# Autodesk Inventor assembly: Rebreather_TMH_Clinical_Test
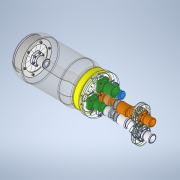
[picture p0: Inventor's stored thumbnail of the model, 180x180]
Saved by Autodesk Inventor 2020 (Build 240168000, 168)
## iProperties
Created: 2021-06-26
Part Number: Rebreather_TMH_Clinical_Test
Document SubType Name: Assembly
Designer: Workshop
Author: Workshop
## Documents named in this file (36)
- D:\Daya 2\Oxy\Bottle D 4 TMH Clinical\3d Files\Rebreather_TMH_Clinical_Test.iam
- D:\Daya 2\Oxy\Bottle D 4 TMH Clinical\3d Files\Container(Sunpet_2L).ipt
- D:\Daya 2\Oxy\Bottle D 4 TMH Clinical\3d Files\Container_Lid(Sunpet_2L).ipt
- D:\Daya 2\Oxy\Bottle D 4 TMH Clinical\3d Files\Bottom_Plate_For_Valve.ipt
- D:\Daya 2\Oxy\Bottle D 4 TMH Clinical\3d Files\Middle_Plate_For_Valve.ipt
- D:\Daya 2\Oxy\Bottle D 4 TMH Clinical\3d Files\Top_Plate_For_Valve.ipt
- C:\Users\Workshop\Documents\Inventor\Content Center Files\R2020\en-US\BS 4168(8)\BS 4168 - M3 x 16(7).ipt
- D:\Daya 2\Oxy\Bottle D 4 TMH Clinical\3d Files\M3_Nylon_Nut.ipt
- D:\Daya 2\Oxy\Bottle D 4 TMH Clinical\3d Files\Silicon_Valve.ipt
- D:\Daya 2\Oxy\Bottle D 4 TMH Clinical\3d Files\Net_Filter.ipt
- D:\Daya 2\Oxy\Bottle D 4 TMH Clinical\3d Files\Net_Retainer.ipt
- D:\Daya 2\Oxy\Bottle D 4 TMH Clinical\3d Files\22M_Airbag_Port_Green.ipt
- D:\Daya 2\Oxy\Bottle D 4 TMH Clinical\3d Files\22M_Exhalation_Port_Orange.ipt
- D:\Daya 2\Oxy\Bottle D 4 TMH Clinical\3d Files\22M_Inhalation_Port_Blue.ipt
- D:\Daya 2\Oxy\Bottle D 4 TMH Clinical\3d Files\22M_PEEP_Port_Female_Green.ipt
- D:\Daya 2\Oxy\Bottle D 4 TMH Clinical\3d Files\22M_Venturi_Port_White.ipt
- D:\Daya 2\Oxy\Bottle D 4 TMH Clinical\3d Files\22M_Diffuser_Port_Sq_Black.ipt
- D:\Daya 2\Oxy\Bottle D 4 TMH Clinical\3d Files\Diffuser_Bottom_Cover.ipt
- D:\Daya 2\Oxy\Bottle D 4 TMH Clinical\3d Files\Diffuser_Filter_Holder.ipt
- D:\Daya 2\Oxy\Bottle D 4 TMH Clinical\3d Files\Diffuser_Top_Cover.ipt
- D:\Daya 2\Oxy\Bottle D 4 TMH Clinical\3d Files\Filter.ipt
- D:\Daya 2\Oxy\Bottle D 4 TMH Clinical\3d Files\22M_Diffuser_Port_Hex_White.ipt
- C:\Users\Workshop\Documents\Inventor\Content Center Files\R2020\en-US\ANSI B18.3.1M(6)\ANSI B18.3.1M - M3x0.5 x 16(1).ipt
- C:\Users\Workshop\Documents\Inventor\Content Center Files\R2020\en-US\ANSI B18.3.1M(6)\ANSI B18.3.1M - M3x0.5 x 45(1).ipt
- D:\Daya 2\Oxy\Bottle D 4 TMH Clinical\3d Files\Connecting_Pipe.ipt
- D:\Daya 2\Oxy\Bottle D 4 TMH Clinical\3d Files\Standalone_Valve_Spacer_Plate.ipt
- D:\Daya 2\Oxy\Bottle D 4 TMH Clinical\3d Files\Standalone_Valve_Cover_Plate.ipt
- D:\Daya 2\Oxy\Bottle D 4 TMH Clinical\3d Files\Standalone_Valve_Base_Plate.ipt
- C:\Users\Workshop\Documents\Inventor\Content Center Files\R2020\en-US\ISO 7091\ISO 7091 - ST 3 - 100 HV.ipt
- C:\Users\Workshop\Documents\Inventor\Content Center Files\R2020\en-US\ANSI B18.3.1M(6)\ANSI B18.3.1M - M3x0.5 x 12(1).ipt
- D:\Daya 2\Oxy\Bottle D 4 TMH Clinical\3d Files\22M_Standalone_Offset_Port_Hex_Female_White.ipt
- D:\Daya 2\Oxy\Bottle D 4 TMH Clinical\3d Files\22M_Standalone_Offset_Port_Hex_Female_Orange.ipt
- D:\Daya 2\Oxy\Bottle D 4 TMH Clinical\3d Files\22M_Standalone_Port_Hex_Lite_Orange.ipt
- D:\Daya 2\Oxy\Bottle D 4 TMH Clinical\3d Files\22M_Standalone_Port_Hex_Lite_White.ipt
- C:\Users\Workshop\Documents\Inventor\Content Center Files\R2020\en-US\ANSI B18.3.1M(6)\ANSI B18.3.1M - M3x0.5 x 25(1).ipt
- D:\Daya 2\Oxy\Bottle D 4 TMH Clinical\3d Files\22M_Male_Female_Adapter.ipt
## Components (118 placed, 35 different names)
1. Container(Sunpet_2L):1 — Mate:1, Mate:2, Flush:1, Insert:1, Insert:48
2. Container_Lid(Sunpet_2L):1 — Insert:1, Mate:3, Insert:2, Insert:3, Insert:11, Insert:12
3. Bottom_Plate_For_Valve:1 — Insert:2, Insert:3, Insert:4, Insert:5, Insert:10
4. Middle_Plate_For_Valve:1 — Insert:4, Insert:5, Insert:6, Insert:7
5. Top_Plate_For_Valve:1 — Insert:6, Insert:7, Insert:8, Insert:9, Angle:1, Insert:15, Insert:16, Insert:17, Insert:18, Insert:19, Insert:20, Insert:21, Insert:22, Insert:23, Insert:24
6. BS 4168 : Part 8 Hexagon socket countersunk and button head screws - Metric series - Metric M3 x 16:1 — Insert:8
7. M3_Nylon_Nut:1 — Insert:9, Angle:1
8. Silicon_Valve:1 — Insert:10
9. Net_Filter:1 — Insert:11, Insert:12, Insert:13, Insert:14, Insert:54, Insert:55
10. Net_Retainer:1 — Insert:13, Insert:14, Insert:25, Insert:26, Insert:56, Insert:57
11. 22M_Airbag_Port_Green:1 — Insert:23, Insert:24
12. 22M_Exhalation_Port_Orange:1 — Insert:17, Insert:18, Insert:49, Insert:50, Insert:51, Insert:52, Insert:107, Angle:9
13. 22M_Inhalation_Port_Blue:1 — Insert:21, Insert:22, Angle:5, Insert:58, Insert:59, Insert:60, Insert:61
14. 22M_PEEP_Port_Female_Green:1 — Insert:19, Insert:20
15. 22M_Venturi_Port_White:1 — Insert:15, Insert:16, Insert:106, Angle:8
16. 22M_Diffuser_Port_Sq_Black:1 — Insert:25, Insert:26, Insert:53, Angle:4, Angle:6, Angle:7
17. Diffuser_Bottom_Cover:1 — Insert:31, Mate:4
18. Diffuser_Filter_Holder:1 — Insert:29, Insert:30, Insert:31, Insert:46, Insert:47
19. Diffuser_Top_Cover:1 — Insert:27, Insert:28, Mate:4, Insert:40, Insert:41, Insert:42, Insert:43, Insert:44, Insert:45, Insert:48
20. Filter:1 — Insert:27, Insert:28, Insert:29, Insert:30, Insert:32, Insert:33
21. 22M_Diffuser_Port_Hex_White:1 — Insert:32, Insert:33, Insert:34, Insert:35, Insert:36, Insert:37, Insert:38, Insert:39, Angle:2, Angle:3, Insert:62
22. Forged Socket Head Cap Screw - Metric M3x0.5 x 16:1 — Insert:34
23. Forged Socket Head Cap Screw - Metric M3x0.5 x 16:2 — Insert:35
24. Forged Socket Head Cap Screw - Metric M3x0.5 x 16:3 — Insert:36
25. Forged Socket Head Cap Screw - Metric M3x0.5 x 16:4 — Insert:37
26. Forged Socket Head Cap Screw - Metric M3x0.5 x 16:5 — Insert:38
27. Forged Socket Head Cap Screw - Metric M3x0.5 x 16:6 — Insert:39
28. Forged Socket Head Cap Screw - Metric M3x0.5 x 16:7 — Insert:40
29. Forged Socket Head Cap Screw - Metric M3x0.5 x 16:8 — Insert:41
30. Forged Socket Head Cap Screw - Metric M3x0.5 x 16:9 — Insert:42
31. Forged Socket Head Cap Screw - Metric M3x0.5 x 16:10 — Insert:43
32. Forged Socket Head Cap Screw - Metric M3x0.5 x 16:11 — Insert:44
33. Forged Socket Head Cap Screw - Metric M3x0.5 x 16:12 — Insert:45
34. Forged Socket Head Cap Screw - Metric M3x0.5 x 45:1 — Insert:49
35. Forged Socket Head Cap Screw - Metric M3x0.5 x 45:2 — Insert:50
36. Forged Socket Head Cap Screw - Metric M3x0.5 x 45:3 — Insert:51
37. Forged Socket Head Cap Screw - Metric M3x0.5 x 45:4 — Insert:52
38. Connecting_Pipe:1 — Insert:62
39. Standalone_Valve_Spacer_Plate:1 — Insert:65, Mate:5, Insert:66, Insert:67
40. Standalone_Valve_Cover_Plate:1 — Insert:68, Insert:69, Insert:74, Insert:93, Mate:9
41. Standalone_Valve_Base_Plate:1 — Insert:63, Insert:65, Mate:5, Insert:91, Insert:92
42. Standalone_Valve_Spacer_Plate:2 — Mate:6, Mate:7, Insert:70, Insert:71, Mate:8
43. Standalone_Valve_Cover_Plate:2 — Insert:72, Insert:73, Insert:75, Insert:88, Insert:89
44. Standalone_Valve_Base_Plate:2 — Insert:64, Mate:6, Mate:7, Insert:90
45. Standalone_Valve_Spacer_Plate:3 — Insert:66, Insert:67, Insert:68, Insert:69
46. Standalone_Valve_Spacer_Plate:4 — Insert:70, Insert:71, Insert:72, Insert:73
47. Silicon_Valve:2 — Insert:63
48. Silicon_Valve:3 — Insert:64
49. ISO 7091 ST 3 - 100 HV:1 — Insert:74, Insert:76
50. ISO 7091 ST 3 - 100 HV:2 — Insert:75, Insert:77
51. Forged Socket Head Cap Screw - Metric M3x0.5 x 12:1 — Insert:76
52. Forged Socket Head Cap Screw - Metric M3x0.5 x 12:2 — Insert:77
53. 22M_Standalone_Offset_Port_Hex_Female_White:1 — Insert:93, Mate:9, Mate:10, Angle:8, Mate:11
54. 22M_Standalone_Offset_Port_Hex_Female_Orange:1 — Insert:88, Insert:89, Mate:12, Angle:9, Mate:13
55. 22M_Standalone_Port_Hex_Lite_Orange:1 — Insert:90, Mate:8, Insert:100, Insert:101, Insert:102, Insert:103, Insert:104, Insert:105
56. 22M_Standalone_Port_Hex_Lite_White:1 — Insert:91, Insert:92, Insert:94, Insert:95, Insert:96, Insert:97, Insert:98, Insert:99
57. Forged Socket Head Cap Screw - Metric M3x0.5 x 25:17 — Insert:94
58. Forged Socket Head Cap Screw - Metric M3x0.5 x 25:18 — Insert:95
59. Forged Socket Head Cap Screw - Metric M3x0.5 x 25:19 — Insert:96
60. Forged Socket Head Cap Screw - Metric M3x0.5 x 25:20 — Insert:97
61. Forged Socket Head Cap Screw - Metric M3x0.5 x 25:21 — Insert:98
62. Forged Socket Head Cap Screw - Metric M3x0.5 x 25:22 — Insert:99
63. Forged Socket Head Cap Screw - Metric M3x0.5 x 25:23 — Insert:100
64. Forged Socket Head Cap Screw - Metric M3x0.5 x 25:24 — Insert:101
65. Forged Socket Head Cap Screw - Metric M3x0.5 x 25:25 — Insert:102
66. Forged Socket Head Cap Screw - Metric M3x0.5 x 25:26 — Insert:103
67. Forged Socket Head Cap Screw - Metric M3x0.5 x 25:27 — Insert:104
68. Forged Socket Head Cap Screw - Metric M3x0.5 x 25:28 — Insert:105
69. 22M_Male_Female_Adapter:1 — Insert:106, Mate:10, Mate:11
70. 22M_Male_Female_Adapter:2 — Insert:107, Mate:12, Mate:13
71. M3_Nylon_Nut:2 — Insert:46, Angle:2
72. M3_Nylon_Nut:3 — Insert:47, Angle:3
73. M3_Nylon_Nut:4
74. M3_Nylon_Nut:5
75. M3_Nylon_Nut:6
76. M3_Nylon_Nut:7
77. M3_Nylon_Nut:8
78. M3_Nylon_Nut:9
79. M3_Nylon_Nut:10
80. M3_Nylon_Nut:11
81. M3_Nylon_Nut:12
82. M3_Nylon_Nut:13
83. M3_Nylon_Nut:14 — Insert:53, Angle:4
84. M3_Nylon_Nut:15
85. M3_Nylon_Nut:16
86. M3_Nylon_Nut:17
87. Forged Socket Head Cap Screw - Metric M3x0.5 x 25:1 — Insert:58
88. M3_Nylon_Nut:18 — Insert:54, Angle:5
89. Forged Socket Head Cap Screw - Metric M3x0.5 x 25:2 — Insert:59
90. M3_Nylon_Nut:19 — Insert:55
91. Forged Socket Head Cap Screw - Metric M3x0.5 x 25:4 — Insert:61
92. M3_Nylon_Nut:20 — Insert:57, Angle:7
93. M3_Nylon_Nut:21 — Insert:56, Angle:6
94. Forged Socket Head Cap Screw - Metric M3x0.5 x 25:3 — Insert:60
95. Forged Socket Head Cap Screw - Metric M3x0.5 x 25:5
96. M3_Nylon_Nut:22
97. Forged Socket Head Cap Screw - Metric M3x0.5 x 25:6
98. M3_Nylon_Nut:23
99. Forged Socket Head Cap Screw - Metric M3x0.5 x 25:7
100. M3_Nylon_Nut:24
101. M3_Nylon_Nut:25
102. Forged Socket Head Cap Screw - Metric M3x0.5 x 25:8
103. Forged Socket Head Cap Screw - Metric M3x0.5 x 25:9
104. M3_Nylon_Nut:26
105. Forged Socket Head Cap Screw - Metric M3x0.5 x 25:10
106. M3_Nylon_Nut:27
107. Forged Socket Head Cap Screw - Metric M3x0.5 x 25:11
108. M3_Nylon_Nut:28
109. M3_Nylon_Nut:29
110. Forged Socket Head Cap Screw - Metric M3x0.5 x 25:12
111. Forged Socket Head Cap Screw - Metric M3x0.5 x 25:13
112. M3_Nylon_Nut:30
113. Forged Socket Head Cap Screw - Metric M3x0.5 x 25:14
114. M3_Nylon_Nut:31
115. Forged Socket Head Cap Screw - Metric M3x0.5 x 25:15
116. M3_Nylon_Nut:32
117. M3_Nylon_Nut:33
118. Forged Socket Head Cap Screw - Metric M3x0.5 x 25:16
## Component patterns: (6 elements, first: M3_Nylon_Nut:2 + M3_Nylon_Nut:3), (4 elements, first: M3_Nylon_Nut:14), (4 elements, first: Forged Socket Head Cap Screw - Metric M3x0.5 x 25:1 + M3_Nylon_Nut:18 + Forged Socket Head Cap Screw - Metric M3x0.5 x 25:2 + M3_Nylon_Nut:19 + Forged Socket Head Cap Screw - Metric M3x0.5 x 25:4 + M3_Nylon_Nut:20 + M3_Nylon_Nut:21 + Forged Socket Head Cap Screw - Metric M3x0.5 x 25:3)
## Relationships (120: Insert 97, Mate 13, Angle 9, Flush 1)
- Mate:1: Container(Sunpet_2L):1
- Mate:2: Container(Sunpet_2L):1
- Flush:1: Container(Sunpet_2L):1
- Insert:1: Container(Sunpet_2L):1 ↔ Container_Lid(Sunpet_2L):1
- Mate:3: Container_Lid(Sunpet_2L):1
- Insert:2: Container_Lid(Sunpet_2L):1 ↔ Bottom_Plate_For_Valve:1
- Insert:3: Container_Lid(Sunpet_2L):1 ↔ Bottom_Plate_For_Valve:1
- Insert:4: Bottom_Plate_For_Valve:1 ↔ Middle_Plate_For_Valve:1
- Insert:5: Bottom_Plate_For_Valve:1 ↔ Middle_Plate_For_Valve:1
- Insert:6: Middle_Plate_For_Valve:1 ↔ Top_Plate_For_Valve:1
- Insert:7: Middle_Plate_For_Valve:1 ↔ Top_Plate_For_Valve:1
- Insert:8: Top_Plate_For_Valve:1 ↔ BS 4168 : Part 8 Hexagon socket countersunk and button head screws - Metric series - Metric M3 x 16:1
- Insert:9: Top_Plate_For_Valve:1 ↔ M3_Nylon_Nut:1
- Angle:1 (0 deg): Top_Plate_For_Valve:1 ↔ M3_Nylon_Nut:1
- Insert:10: Bottom_Plate_For_Valve:1 ↔ Silicon_Valve:1
- Insert:11: Container_Lid(Sunpet_2L):1 ↔ Net_Filter:1
- Insert:12: Container_Lid(Sunpet_2L):1 ↔ Net_Filter:1
- Insert:13: Net_Filter:1 ↔ Net_Retainer:1
- Insert:14: Net_Filter:1 ↔ Net_Retainer:1
- Insert:15: Top_Plate_For_Valve:1 ↔ 22M_Venturi_Port_White:1
- Insert:16: Top_Plate_For_Valve:1 ↔ 22M_Venturi_Port_White:1
- Insert:17: Top_Plate_For_Valve:1 ↔ 22M_Exhalation_Port_Orange:1
- Insert:18: Top_Plate_For_Valve:1 ↔ 22M_Exhalation_Port_Orange:1
- Insert:19: Top_Plate_For_Valve:1 ↔ 22M_PEEP_Port_Female_Green:1
- Insert:20: Top_Plate_For_Valve:1 ↔ 22M_PEEP_Port_Female_Green:1
- Insert:21: Top_Plate_For_Valve:1 ↔ 22M_Inhalation_Port_Blue:1
- Insert:22: Top_Plate_For_Valve:1 ↔ 22M_Inhalation_Port_Blue:1
- Insert:23: Top_Plate_For_Valve:1 ↔ 22M_Airbag_Port_Green:1
- Insert:24: Top_Plate_For_Valve:1 ↔ 22M_Airbag_Port_Green:1
- Insert:25: Net_Retainer:1 ↔ 22M_Diffuser_Port_Sq_Black:1
- Insert:26: Net_Retainer:1 ↔ 22M_Diffuser_Port_Sq_Black:1
- Insert:27: Diffuser_Top_Cover:1 ↔ Filter:1
- Insert:28: Diffuser_Top_Cover:1 ↔ Filter:1
- Insert:29: Diffuser_Filter_Holder:1 ↔ Filter:1
- Insert:30: Diffuser_Filter_Holder:1 ↔ Filter:1
- Insert:31: Diffuser_Bottom_Cover:1 ↔ Diffuser_Filter_Holder:1
- Mate:4: Diffuser_Bottom_Cover:1 ↔ Diffuser_Top_Cover:1
- Insert:32: Filter:1 ↔ 22M_Diffuser_Port_Hex_White:1
- Insert:33: Filter:1 ↔ 22M_Diffuser_Port_Hex_White:1
- Insert:34: 22M_Diffuser_Port_Hex_White:1 ↔ Forged Socket Head Cap Screw - Metric M3x0.5 x 16:1
- Insert:35: 22M_Diffuser_Port_Hex_White:1 ↔ Forged Socket Head Cap Screw - Metric M3x0.5 x 16:2
- Insert:36: 22M_Diffuser_Port_Hex_White:1 ↔ Forged Socket Head Cap Screw - Metric M3x0.5 x 16:3
- Insert:37: 22M_Diffuser_Port_Hex_White:1 ↔ Forged Socket Head Cap Screw - Metric M3x0.5 x 16:4
- Insert:38: 22M_Diffuser_Port_Hex_White:1 ↔ Forged Socket Head Cap Screw - Metric M3x0.5 x 16:5
- Insert:39: 22M_Diffuser_Port_Hex_White:1 ↔ Forged Socket Head Cap Screw - Metric M3x0.5 x 16:6
- Insert:40: Diffuser_Top_Cover:1 ↔ Forged Socket Head Cap Screw - Metric M3x0.5 x 16:7
- Insert:41: Diffuser_Top_Cover:1 ↔ Forged Socket Head Cap Screw - Metric M3x0.5 x 16:8
- Insert:42: Diffuser_Top_Cover:1 ↔ Forged Socket Head Cap Screw - Metric M3x0.5 x 16:9
- Insert:43: Diffuser_Top_Cover:1 ↔ Forged Socket Head Cap Screw - Metric M3x0.5 x 16:10
- Insert:44: Diffuser_Top_Cover:1 ↔ Forged Socket Head Cap Screw - Metric M3x0.5 x 16:11
- Insert:45: Diffuser_Top_Cover:1 ↔ Forged Socket Head Cap Screw - Metric M3x0.5 x 16:12
- Insert:46: Diffuser_Filter_Holder:1 ↔ M3_Nylon_Nut:2
- Insert:47: Diffuser_Filter_Holder:1 ↔ M3_Nylon_Nut:3
- Angle:2 (0 deg): 22M_Diffuser_Port_Hex_White:1 ↔ M3_Nylon_Nut:2
- Angle:3 (0 deg): 22M_Diffuser_Port_Hex_White:1 ↔ M3_Nylon_Nut:3
- Insert:48: Container(Sunpet_2L):1 ↔ Diffuser_Top_Cover:1
- Insert:49: 22M_Exhalation_Port_Orange:1 ↔ Forged Socket Head Cap Screw - Metric M3x0.5 x 45:1
- Insert:50: 22M_Exhalation_Port_Orange:1 ↔ Forged Socket Head Cap Screw - Metric M3x0.5 x 45:2
- Insert:51: 22M_Exhalation_Port_Orange:1 ↔ Forged Socket Head Cap Screw - Metric M3x0.5 x 45:3
- Insert:52: 22M_Exhalation_Port_Orange:1 ↔ Forged Socket Head Cap Screw - Metric M3x0.5 x 45:4
- Insert:53: 22M_Diffuser_Port_Sq_Black:1 ↔ M3_Nylon_Nut:14
- Angle:4 (0 deg): 22M_Diffuser_Port_Sq_Black:1 ↔ M3_Nylon_Nut:14
- Insert:54: Net_Filter:1 ↔ M3_Nylon_Nut:18
- Angle:5 (0 deg): 22M_Inhalation_Port_Blue:1 ↔ M3_Nylon_Nut:18
- Insert:55: Net_Filter:1 ↔ M3_Nylon_Nut:19
- Insert:56: Net_Retainer:1 ↔ M3_Nylon_Nut:21
- Insert:57: Net_Retainer:1 ↔ M3_Nylon_Nut:20
- Angle:6 (0 deg): 22M_Diffuser_Port_Sq_Black:1 ↔ M3_Nylon_Nut:21
- Angle:7 (0 deg): 22M_Diffuser_Port_Sq_Black:1 ↔ M3_Nylon_Nut:20
- Insert:58: 22M_Inhalation_Port_Blue:1 ↔ Forged Socket Head Cap Screw - Metric M3x0.5 x 25:1
- Insert:59: 22M_Inhalation_Port_Blue:1 ↔ Forged Socket Head Cap Screw - Metric M3x0.5 x 25:2
- Insert:60: 22M_Inhalation_Port_Blue:1 ↔ Forged Socket Head Cap Screw - Metric M3x0.5 x 25:3
- Insert:61: 22M_Inhalation_Port_Blue:1 ↔ Forged Socket Head Cap Screw - Metric M3x0.5 x 25:4
- Insert:62: 22M_Diffuser_Port_Hex_White:1 ↔ Connecting_Pipe:1
- Insert:63: Standalone_Valve_Base_Plate:1 ↔ Silicon_Valve:2
- Insert:64: Standalone_Valve_Base_Plate:2 ↔ Silicon_Valve:3
- Insert:65: Standalone_Valve_Spacer_Plate:1 ↔ Standalone_Valve_Base_Plate:1
- Mate:5: Standalone_Valve_Spacer_Plate:1 ↔ Standalone_Valve_Base_Plate:1
- Insert:66: Standalone_Valve_Spacer_Plate:1 ↔ Standalone_Valve_Spacer_Plate:3
- Insert:67: Standalone_Valve_Spacer_Plate:1 ↔ Standalone_Valve_Spacer_Plate:3
- Insert:68: Standalone_Valve_Cover_Plate:1 ↔ Standalone_Valve_Spacer_Plate:3
- Insert:69: Standalone_Valve_Cover_Plate:1 ↔ Standalone_Valve_Spacer_Plate:3
- Mate:6: Standalone_Valve_Spacer_Plate:2 ↔ Standalone_Valve_Base_Plate:2
- Mate:7: Standalone_Valve_Spacer_Plate:2 ↔ Standalone_Valve_Base_Plate:2
- Insert:70: Standalone_Valve_Spacer_Plate:2 ↔ Standalone_Valve_Spacer_Plate:4
- Insert:71: Standalone_Valve_Spacer_Plate:2 ↔ Standalone_Valve_Spacer_Plate:4
- Insert:72: Standalone_Valve_Cover_Plate:2 ↔ Standalone_Valve_Spacer_Plate:4
- Insert:73: Standalone_Valve_Cover_Plate:2 ↔ Standalone_Valve_Spacer_Plate:4
- Insert:74: Standalone_Valve_Cover_Plate:1 ↔ ISO 7091 ST 3 - 100 HV:1
- Insert:75: Standalone_Valve_Cover_Plate:2 ↔ ISO 7091 ST 3 - 100 HV:2
- Insert:76: ISO 7091 ST 3 - 100 HV:1 ↔ Forged Socket Head Cap Screw - Metric M3x0.5 x 12:1
- Insert:77: ISO 7091 ST 3 - 100 HV:2 ↔ Forged Socket Head Cap Screw - Metric M3x0.5 x 12:2
- Insert:88: Standalone_Valve_Cover_Plate:2 ↔ 22M_Standalone_Offset_Port_Hex_Female_Orange:1
- Insert:89: Standalone_Valve_Cover_Plate:2 ↔ 22M_Standalone_Offset_Port_Hex_Female_Orange:1
- Insert:90: Standalone_Valve_Base_Plate:2 ↔ 22M_Standalone_Port_Hex_Lite_Orange:1
- Mate:8: Standalone_Valve_Spacer_Plate:2 ↔ 22M_Standalone_Port_Hex_Lite_Orange:1
- Insert:91: Standalone_Valve_Base_Plate:1 ↔ 22M_Standalone_Port_Hex_Lite_White:1
- Insert:92: Standalone_Valve_Base_Plate:1 ↔ 22M_Standalone_Port_Hex_Lite_White:1
- Insert:93: Standalone_Valve_Cover_Plate:1 ↔ 22M_Standalone_Offset_Port_Hex_Female_White:1
- Mate:9: Standalone_Valve_Cover_Plate:1 ↔ 22M_Standalone_Offset_Port_Hex_Female_White:1
- Insert:94: 22M_Standalone_Port_Hex_Lite_White:1 ↔ Forged Socket Head Cap Screw - Metric M3x0.5 x 25:17
- Insert:95: 22M_Standalone_Port_Hex_Lite_White:1 ↔ Forged Socket Head Cap Screw - Metric M3x0.5 x 25:18
- Insert:96: 22M_Standalone_Port_Hex_Lite_White:1 ↔ Forged Socket Head Cap Screw - Metric M3x0.5 x 25:19
- Insert:97: 22M_Standalone_Port_Hex_Lite_White:1 ↔ Forged Socket Head Cap Screw - Metric M3x0.5 x 25:20
- Insert:98: 22M_Standalone_Port_Hex_Lite_White:1 ↔ Forged Socket Head Cap Screw - Metric M3x0.5 x 25:21
- Insert:99: 22M_Standalone_Port_Hex_Lite_White:1 ↔ Forged Socket Head Cap Screw - Metric M3x0.5 x 25:22
- Insert:100: 22M_Standalone_Port_Hex_Lite_Orange:1 ↔ Forged Socket Head Cap Screw - Metric M3x0.5 x 25:23
- Insert:101: 22M_Standalone_Port_Hex_Lite_Orange:1 ↔ Forged Socket Head Cap Screw - Metric M3x0.5 x 25:24
- Insert:102: 22M_Standalone_Port_Hex_Lite_Orange:1 ↔ Forged Socket Head Cap Screw - Metric M3x0.5 x 25:25
- Insert:103: 22M_Standalone_Port_Hex_Lite_Orange:1 ↔ Forged Socket Head Cap Screw - Metric M3x0.5 x 25:26
- Insert:104: 22M_Standalone_Port_Hex_Lite_Orange:1 ↔ Forged Socket Head Cap Screw - Metric M3x0.5 x 25:27
- Insert:105: 22M_Standalone_Port_Hex_Lite_Orange:1 ↔ Forged Socket Head Cap Screw - Metric M3x0.5 x 25:28
- Insert:106 (3 mm): 22M_Venturi_Port_White:1 ↔ 22M_Male_Female_Adapter:1
- Insert:107 (-3 mm): 22M_Exhalation_Port_Orange:1 ↔ 22M_Male_Female_Adapter:2
- Mate:10: 22M_Standalone_Offset_Port_Hex_Female_White:1 ↔ 22M_Male_Female_Adapter:1
- Angle:8 (0 deg): 22M_Venturi_Port_White:1 ↔ 22M_Standalone_Offset_Port_Hex_Female_White:1
- Mate:11 (-4 mm): 22M_Standalone_Offset_Port_Hex_Female_White:1 ↔ 22M_Male_Female_Adapter:1
- Mate:12: 22M_Standalone_Offset_Port_Hex_Female_Orange:1 ↔ 22M_Male_Female_Adapter:2
- Angle:9 (0 deg): 22M_Exhalation_Port_Orange:1 ↔ 22M_Standalone_Offset_Port_Hex_Female_Orange:1
- Mate:13 (-4 mm): 22M_Standalone_Offset_Port_Hex_Female_Orange:1 ↔ 22M_Male_Female_Adapter:2
